# Autodesk Inventor assembly: Cabin Assembly
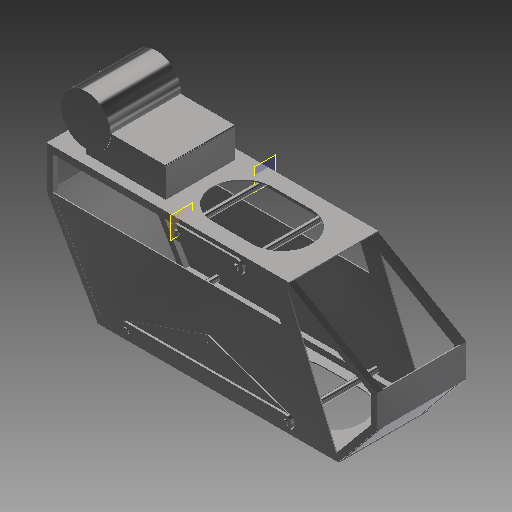
[picture p0: Inventor's stored thumbnail of the model, 512x512]
Saved by Autodesk Inventor 2019 (Build 230136000, 136)
## iProperties
Created: 2019-08-25
Part Number: Cabin Assembly
Document SubType Name: Assembly
Designer: DIBYOJYOTI
Mass: 1511.06 g
Surface Area: 3025.21 cm^2
Volume: 192.662 cm^3
Density: 7.8431 g/cm^3
Author: DIBYOJYOTI
## Documents named in this file (8)
- D:\Autocad\Cabin Assembly.iam
- D:\Autocad\Upper Rod extended Spider Crab.ipt
- D:\Autocad\Cabin Roof.ipt
- D:\Autocad\Cabin front panel.ipt
- D:\Autocad\Cabin Back Panel.ipt
- D:\Autocad\Battery Box.ipt
- D:\Autocad\Cabin Wall Assembly.iam
- D:\Autocad\Cabin Wall Assembly_MIR.iam
## Components (11 placed, 7 different names)
1. Upper Rod extended Spider Crab:1 — Insert:11
2. Upper Rod extended Spider Crab:2 — Insert:7, Insert:9
3. Upper Rod extended Spider Crab:3 — Insert:8, Insert:10
4. Upper Rod extended Spider Crab:4 — Insert:12
5. Cabin Roof:1 — Flush:10, Flush:12, Flush:15, Flush:16, Flush:17, Flush:18
6. Cabin Roof:2 — Flush:18, Flush:19, Flush:20
7. Cabin front panel:1 — Flush:13, Flush:14
8. Cabin Back Panel:1 — Rigid:1
9. Battery Box:1 — Flush:10, Flush:12
10. Cabin Wall Assembly:1 [sub-assembly] — Insert:7, Insert:8, Flush:15, Flush:16, Flush:17
11. Cabin Wall Assembly_MIR:1 [sub-assembly] — Insert:9, Insert:10, Flush:13, Flush:14, Flush:19, Flush:20, Insert:11, Insert:12, Rigid:1
## Relationships (17: Flush 10, Insert 6, WeldJoint 1)
- Flush:10: Cabin Roof:1 ↔ Battery Box:1
- Flush:12 (30 mm): Cabin Roof:1 ↔ Battery Box:1
- Insert:7 (2 mm): Upper Rod extended Spider Crab:2 ↔ Cabin Wall Assembly:1
- Insert:8 (1 mm): Upper Rod extended Spider Crab:3 ↔ Cabin Wall Assembly:1
- Insert:9 (2 mm): Upper Rod extended Spider Crab:2 ↔ Cabin Wall Assembly_MIR:1
- Insert:10 (1 mm): Upper Rod extended Spider Crab:3 ↔ Cabin Wall Assembly_MIR:1
- Flush:13: Cabin front panel:1 ↔ Cabin Wall Assembly_MIR:1
- Flush:14 (6 mm): Cabin front panel:1 ↔ Cabin Wall Assembly_MIR:1
- Flush:15 (-1 mm): Cabin Roof:1 ↔ Cabin Wall Assembly:1
- Flush:16: Cabin Roof:1 ↔ Cabin Wall Assembly:1
- Flush:17: Cabin Roof:1 ↔ Cabin Wall Assembly:1
- Flush:18 (131 mm): Cabin Roof:1 ↔ Cabin Roof:2
- Flush:19 (75 mm): Cabin Roof:2 ↔ Cabin Wall Assembly_MIR:1
- Flush:20 (50.607 mm): Cabin Roof:2 ↔ Cabin Wall Assembly_MIR:1
- Insert:11 (2 mm): Upper Rod extended Spider Crab:1 ↔ Cabin Wall Assembly_MIR:1
- Insert:12 (1 mm): Upper Rod extended Spider Crab:4 ↔ Cabin Wall Assembly_MIR:1
- Rigid:1 [WeldJoint]: Cabin Back Panel:1 ↔ Cabin Wall Assembly_MIR:1
